# Autodesk Inventor assembly: Sistema de extracción
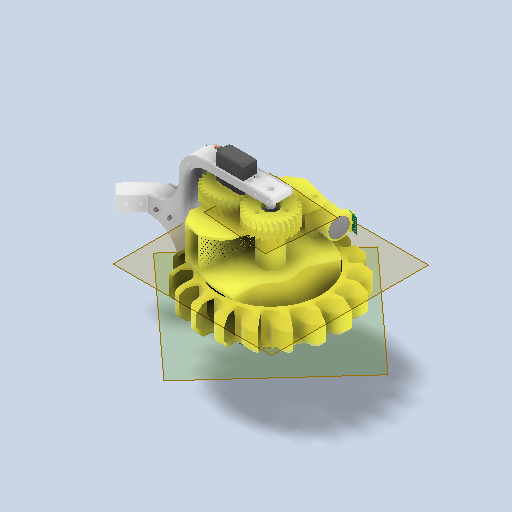
[picture p0: Inventor's stored thumbnail of the model, 512x512]
Saved by Autodesk Inventor 2022 (Build 260153000, 153)
## iProperties
Created: 2021-10-11
Part Number: Sistema de extracción
Document SubType Name: Assembly
Designer: juanp
Author: juanp
## Documents named in this file (16)
- C:\Users\juanp\Desktop\Robocol\Sistema de extracción\Sistema de extracción.iam
- C:\Users\juanp\Desktop\Robocol\Sistema de extracción\Solid1.ipt
- C:\Users\juanp\Desktop\Robocol\Sistema de extracción\Solid2.ipt
- C:\Users\juanp\Desktop\Robocol\Sistema de extracción\Solid7.ipt
- C:\Users\juanp\Desktop\Robocol\Sistema de extracción\Recursos\Servo MG996R\Servo Motor MG996R.iam
- C:\Users\juanp\Desktop\Robocol\Sistema de extracción\Brazo\Soporte.ipt
- C:\Users\juanp\Desktop\Robocol\Sistema de extracción\piñon colector.ipt
- C:\Users\juanp\Desktop\Robocol\Sistema de extracción\piñon rueda.ipt
- C:\Users\juanp\Desktop\Robocol\Sistema de extracción\Recursos\Sensores\sensorhumedad.ipt
- C:\Users\juanp\Desktop\Robocol\Sistema de extracción\Recursos\Sensores\tempsensor.ipt
- C:\Users\juanp\Desktop\Robocol\Sistema de extracción\Solid13.ipt
- C:\Users\juanp\Desktop\Robocol\Sistema de extracción\Solid17_1.ipt
- C:\Users\juanp\Desktop\Robocol\Sistema de extracción\Recursos\Motor DC\Motor DC.ipt
- C:\Users\juanp\Desktop\Robocol\Sistema de extracción\Espaciadores.ipt
- C:\Users\juanp\Desktop\Robocol\Sistema de extracción\Recursos\Sensores\GY-521.ipt
- C:\Users\juanp\Documents\Inventor\Content Center Files\R2022\en-US\AS 1427(00)\AS 1427 - M5 x 35(4).ipt
## Components (17 placed, 15 different names)
1. Solid1:1 — Symmetry:1, Flush:2, Mate:12, Mate:13
2. Solid2:1 — Mate:13, Mate:14, Mate:20, Mate:25, Mate:26, Mate:27, Flush:3, Flush:4, Mate:28, Mate:29, Mate:30, Mate:31, Mate:32
3. Solid7:1 — Mate:4, Flush:1, Symmetry:1, Mate:14
4. Servo Motor MG996R:1 [sub-assembly] — Mate:1, Mate:2, Mate:3, Mate:5, Mate:6
5. Soporte:1 — Mate:1, Mate:2, Mate:3, Mate:4, Mate:7, Angle:1, Mate:12, Mate:23, Mate:24, Mate:35, Mate:36, Mate:40, Mate:41, Mate:42, Mate:43
6. piñon colector:1 — Mate:5, Mate:6, Flush:1
7. Servo Motor MG996R:2 [sub-assembly] — Mate:7, Mate:10, Mate:11, Mate:23, Mate:24
8. piñon rueda:1 — Mate:10, Mate:11, Flush:2
9. sensorhumedad:1 — Mate:25, Mate:26, Mate:31
10. tempsensor:1 — Mate:20, Mate:32
11. Solid13:1 — Mate:28, Mate:29, Mate:30
12. Solid17_1:1 — Mate:27, Flush:3, Flush:4, Mate:33, Mate:34, Mate:37, Mate:38, Mate:39
13. Espaciadores:1 — Mate:35, Mate:36
14. Motor DC:1 — Mate:33, Mate:34
15. GY-521:1 — Mate:37, Mate:38, Mate:39
16. AS 1427 - Metric M5 x 35:1 — Mate:40, Mate:42
17. AS 1427 - Metric M5 x 35:2 — Mate:41, Mate:43
## Relationships (40: Mate 34, Flush 4, Symmetry 1, Angle 1)
- Mate:1: Servo Motor MG996R:1 ↔ Soporte:1
- Mate:2: Servo Motor MG996R:1 ↔ Soporte:1
- Mate:3: Servo Motor MG996R:1 ↔ Soporte:1
- Mate:4: Solid7:1 ↔ Soporte:1
- Mate:5: Servo Motor MG996R:1 ↔ piñon colector:1
- Mate:6: Servo Motor MG996R:1 ↔ piñon colector:1
- Flush:1: Solid7:1 ↔ piñon colector:1
- Symmetry:1: Solid1:1 ↔ Solid7:1
- Mate:7: Soporte:1 ↔ Servo Motor MG996R:2
- Mate:10: Servo Motor MG996R:2 ↔ piñon rueda:1
- Mate:11: Servo Motor MG996R:2 ↔ piñon rueda:1
- Angle:1 (180 deg): Soporte:1
- Flush:2: Solid1:1 ↔ piñon rueda:1
- Mate:12: Solid1:1 ↔ Soporte:1
- Mate:13: Solid1:1 ↔ Solid2:1
- Mate:14: Solid2:1 ↔ Solid7:1
- Mate:20: Solid2:1 ↔ tempsensor:1
- Mate:23: Soporte:1 ↔ Servo Motor MG996R:2
- Mate:24: Soporte:1 ↔ Servo Motor MG996R:2
- Mate:25: Solid2:1 ↔ sensorhumedad:1
- Mate:26: Solid2:1 ↔ sensorhumedad:1
- Mate:27: Solid2:1 ↔ Solid17_1:1
- Flush:3: Solid2:1 ↔ Solid17_1:1
- Flush:4: Solid2:1 ↔ Solid17_1:1
- Mate:28 (0.2 mm): Solid2:1 ↔ Solid13:1
- Mate:29: Solid2:1 ↔ Solid13:1
- Mate:30: Solid2:1 ↔ Solid13:1
- Mate:31: Solid2:1 ↔ sensorhumedad:1
- Mate:32: Solid2:1 ↔ tempsensor:1
- Mate:33: Solid17_1:1 ↔ Motor DC:1
- Mate:34: Solid17_1:1 ↔ Motor DC:1
- Mate:35: Soporte:1 ↔ Espaciadores:1
- Mate:36: Soporte:1 ↔ Espaciadores:1
- Mate:37: Solid17_1:1 ↔ GY-521:1
- Mate:38: Solid17_1:1 ↔ GY-521:1
- Mate:39: Solid17_1:1 ↔ GY-521:1
- Mate:40: Soporte:1 ↔ AS 1427 - Metric M5 x 35:1
- Mate:41: Soporte:1 ↔ AS 1427 - Metric M5 x 35:2
- Mate:42: Soporte:1 ↔ AS 1427 - Metric M5 x 35:1
- Mate:43: Soporte:1 ↔ AS 1427 - Metric M5 x 35:2
